# Autodesk Inventor assembly: dribler
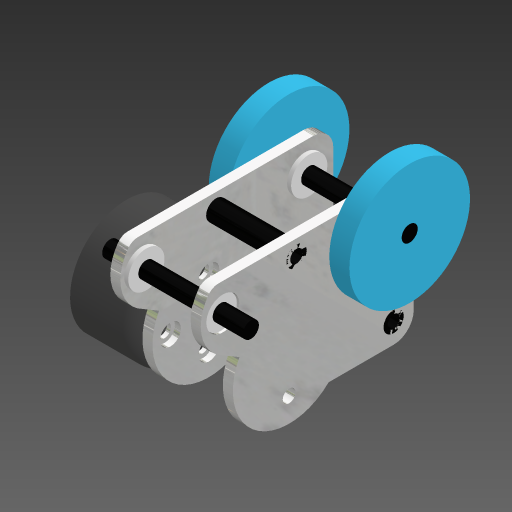
[picture p0: Inventor's stored thumbnail of the model, 512x512]
Saved by Autodesk Inventor 2023 (Build 270158000, 158)
## iProperties
Created: 2025-06-01
Part Number: dribler
Document SubType Name: Assembly
Designer: daa
Author: daa
## Documents named in this file (8)
- C:\Users\daa\Documents\DASH_\Dash-V1\Dribler_v2\dribler.iam
- C:\Users\daa\Documents\DASH_\Dash-V1\Dribler_v2\drib_lef.ipt
- C:\Users\daa\Documents\DASH_\Dash-V1\Dribler_v2\drib_rig.ipt
- C:\Users\daa\Documents\DASH_\Dash-V1\Dribler_v2\motor_c2822.ipt
- C:\Users\daa\Documents\DASH_\Dash-V1\Dribler_v2\bearing.ipt
- C:\Users\daa\Documents\DASH_\Dash-V1\Dribler_v2\rack.ipt
- C:\Users\daa\Documents\DASH_\Dash-V1\Dribler_v2\axis.ipt
- C:\Users\daa\Documents\kolles.ipt
## Components (13 placed, 7 different names)
1. drib_lef:1 — С поворотом:1, С поворотом:3, С поворотом:6
2. drib_rig:1 — С поворотом:1, С поворотом:2, С поворотом:4, С поворотом:5, С поворотом:7, С поворотом:8
3. motor_c2822:1 — С поворотом:2
4. bearing:1 — С поворотом:3
5. bearing:2 — С поворотом:4, С поворотом:10
6. bearing:3 — С поворотом:6
7. bearing:4 — С поворотом:5, С поворотом:9
8. rack:1 — С поворотом:7
9. rack:2 — С поворотом:8
10. axis:1 — С поворотом:9, Жесткий:1, Жесткий:2
11. kolles:1 — Жесткий:2
12. kolles:2 — Жесткий:1
13. axis:2 — С поворотом:10
## Relationships (12: RevoluteJoint 10, WeldJoint 2)
- С поворотом:1 [RevoluteJoint] (20 mm): drib_lef:1 ↔ drib_rig:1
- С поворотом:2 [RevoluteJoint] (-6 mm): drib_rig:1 ↔ motor_c2822:1
- С поворотом:3 [RevoluteJoint] (-2 mm): drib_lef:1 ↔ bearing:1
- С поворотом:4 [RevoluteJoint] (2 mm): drib_rig:1 ↔ bearing:2
- С поворотом:5 [RevoluteJoint] (2 mm): drib_rig:1 ↔ bearing:4
- С поворотом:6 [RevoluteJoint] (-2 mm): drib_lef:1 ↔ bearing:3
- С поворотом:7 [RevoluteJoint]: drib_rig:1 ↔ rack:1
- С поворотом:8 [RevoluteJoint]: drib_rig:1 ↔ rack:2
- С поворотом:9 [RevoluteJoint] (10 mm): bearing:4 ↔ axis:1
- Жесткий:1 [WeldJoint]: axis:1 ↔ kolles:2
- Жесткий:2 [WeldJoint]: axis:1 ↔ kolles:1
- С поворотом:10 [RevoluteJoint] (6 mm): bearing:2 ↔ axis:2
